# Autodesk Inventor assembly: Assy_curve_module
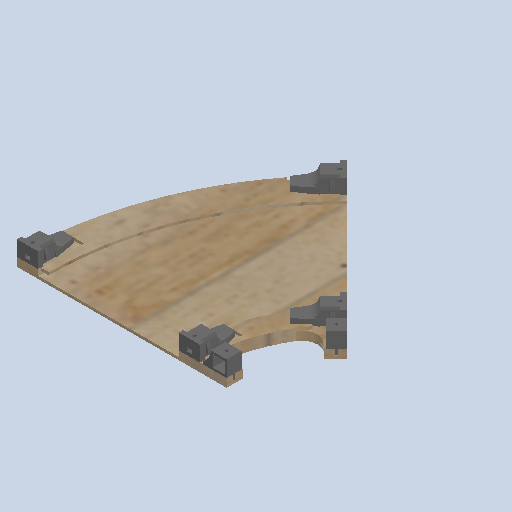
[picture p0: Inventor's stored thumbnail of the model, 512x512]
Saved by Autodesk Inventor 2024.1 (Build 281209000, 209)
## iProperties
Created: 2025-09-28
Part Number: Assy_curve_module
Document SubType Name: Assembly
Designer: hibik
Author: hibik
## Documents named in this file (8)
- C:\Users\hibik\Documents\Robomech\conveyer\curve_module\Assy_curve_module.iam
- C:\Users\hibik\Documents\Robomech\conveyer\curve_module\base.ipt
- C:\Users\hibik\Documents\Robomech\conveyer\curve_module\back_under.ipt
- C:\Users\hibik\Documents\Robomech\conveyer\curve_module\back_upper.ipt
- C:\Users\hibik\Documents\Robomech\conveyer\curve_module\front_under.ipt
- C:\Users\hibik\Documents\Robomech\conveyer\curve_module\front_upper.ipt
- C:\Users\hibik\Documents\Robomech\conveyer\connector_module\connector_male.ipt
- C:\Users\hibik\Documents\Robomech\conveyer\connector_module\position_setter_normal.ipt
## Components (11 placed, 7 different names)
1. base:1 — 挿入:3, 挿入:5
2. front_under:1 — 挿入:3, 挿入:4, 角度:3, 挿入:11, 角度:11, 挿入:12, 角度:12
3. front_upper:1 — 挿入:4, 角度:4
4. position_setter_normal:1 — 挿入:9, 角度:9
5. connector_male:2 — 挿入:7, 角度:7
6. back_under:1 — 挿入:5, 挿入:6, 角度:5, 挿入:7, 角度:7, 挿入:8, 角度:8, 挿入:9, 角度:9, 挿入:10, 角度:10
7. back_upper:1 — 挿入:6, 角度:6
8. connector_male:3 — 挿入:8, 角度:8
9. connector_male:4 — 挿入:11, 角度:11
10. connector_male:5 — 挿入:12, 角度:12
11. position_setter_normal:2 — 挿入:10, 角度:10
## Relationships (20: Insert 10, Angle 10)
- 挿入:3 [Insert]: base:1 ↔ front_under:1
- 挿入:4 [Insert]: front_under:1 ↔ front_upper:1
- 角度:3 [Angle] (0 deg): front_under:1
- 角度:4 [Angle] (0 deg): front_upper:1
- 挿入:5 [Insert]: base:1 ↔ back_under:1
- 挿入:6 [Insert]: back_under:1 ↔ back_upper:1
- 角度:5 [Angle] (0 deg): back_under:1
- 角度:6 [Angle] (0 deg): back_upper:1
- 挿入:7 [Insert]: connector_male:2 ↔ back_under:1
- 角度:7 [Angle] (0 deg): connector_male:2 ↔ back_under:1
- 挿入:8 [Insert]: back_under:1 ↔ connector_male:3
- 角度:8 [Angle] (0 deg): back_under:1 ↔ connector_male:3
- 挿入:9 [Insert]: position_setter_normal:1 ↔ back_under:1
- 角度:9 [Angle] (0 deg): position_setter_normal:1 ↔ back_under:1
- 挿入:10 [Insert]: back_under:1 ↔ position_setter_normal:2
- 角度:10 [Angle] (0 deg): back_under:1 ↔ position_setter_normal:2
- 挿入:11 [Insert]: front_under:1 ↔ connector_male:4
- 角度:11 [Angle] (0 deg): front_under:1 ↔ connector_male:4
- 挿入:12 [Insert]: front_under:1 ↔ connector_male:5
- 角度:12 [Angle] (0 deg): front_under:1 ↔ connector_male:5
